# Autodesk Inventor assembly: Additional_Building
(part 2 of 2)
- Flush:52: Walls:1 ↔ Stud_Between_Top_Plate_And_Rafter_3:1
- Flush:53: Walls:1 ↔ Stud_Between_Top_Plate_And_Rafter_3:1
- Mate:71: Walls:1 ↔ Stud_Between_Top_Plate_And_Rafter_4:1
- Flush:54: Walls:1 ↔ Stud_Between_Top_Plate_And_Rafter_4:1
- Flush:55: Walls:1 ↔ Stud_Between_Top_Plate_And_Rafter_4:1
- Mate:72: Walls:1 ↔ Stud_Between_Top_Plate_And_Rafter_5:1
- Flush:56: Walls:1 ↔ Stud_Between_Top_Plate_And_Rafter_5:1
- Flush:57: Walls:1 ↔ Stud_Between_Top_Plate_And_Rafter_5:1
- Mate:73: Walls:1 ↔ Stud_Between_Top_Plate_And_Rafter_6:1
- Flush:58: Walls:1 ↔ Stud_Between_Top_Plate_And_Rafter_6:1
- Flush:59: Walls:1 ↔ Stud_Between_Top_Plate_And_Rafter_6:1
- Mate:74: Walls:1 ↔ Stud_Between_Top_Plate_And_Rafter_7:1
- Flush:60: Walls:1 ↔ Stud_Between_Top_Plate_And_Rafter_7:1
- Flush:61: Walls:1 ↔ Stud_Between_Top_Plate_And_Rafter_7:1
- Mate:75: Walls:1 ↔ Stud_Between_Top_Plate_And_Rafter_8:1
- Flush:62: Walls:1 ↔ Stud_Between_Top_Plate_And_Rafter_8:1
- Flush:63: Walls:1 ↔ Stud_Between_Top_Plate_And_Rafter_8:1
- Mate:76: Walls:1 ↔ Stud_Between_Top_Plate_And_Rafter_9:1
- Mate:77: Truss:1 ↔ Stud_Between_Top_Plate_And_Rafter_9:1
- Flush:64: Walls:1 ↔ Stud_Between_Top_Plate_And_Rafter_9:1
- Mate:78: Walls:1 ↔ Stud_With_Height_41.707_Inches:1
- Mate:79: Truss:1 ↔ Stud_With_Height_41.707_Inches:1
- Mate:80: Stud_Between_Top_Plate_And_Rafter_9:1 ↔ Stud_With_Height_41.707_Inches:1
- Mate:81: Truss:3 ↔ Support_For_Ceiling:1
- Flush:65: Truss:1 ↔ Support_For_Ceiling:1
- Flush:66: Stud_Between_Top_Plate_And_Rafter_1:1 ↔ Support_For_Ceiling:1
- Mate:82: Truss:3 ↔ Support_For_Ceiling:2
- Flush:67: Truss:1 ↔ Support_For_Ceiling:2
- Flush:68: Stud_Between_Top_Plate_And_Rafter_2:1 ↔ Support_For_Ceiling:2
- Mate:83: Truss:3 ↔ Support_For_Ceiling:3
- Flush:69: Truss:1 ↔ Support_For_Ceiling:3
- Flush:70: Stud_Between_Top_Plate_And_Rafter_3:1 ↔ Support_For_Ceiling:3
- Mate:84: Truss:3 ↔ Support_For_Ceiling:4
- Flush:71: Truss:1 ↔ Support_For_Ceiling:4
- Flush:72: Stud_Between_Top_Plate_And_Rafter_4:1 ↔ Support_For_Ceiling:4
- Mate:85: Truss:3 ↔ Support_For_Ceiling:5
- Flush:73: Truss:1 ↔ Support_For_Ceiling:5
- Flush:74: Stud_Between_Top_Plate_And_Rafter_5:1 ↔ Support_For_Ceiling:5
- Mate:86: Truss:3 ↔ Support_For_Ceiling:6
- Flush:75: Truss:1 ↔ Support_For_Ceiling:6
- Flush:76: Stud_Between_Top_Plate_And_Rafter_6:1 ↔ Support_For_Ceiling:6
- Mate:87: Truss:3 ↔ Support_For_Ceiling:7
- Flush:77: Truss:1 ↔ Support_For_Ceiling:7
- Flush:78: Stud_Between_Top_Plate_And_Rafter_7:1 ↔ Support_For_Ceiling:7
- Mate:88: Truss:3 ↔ Support_For_Ceiling:8
- Flush:79: Truss:1 ↔ Support_For_Ceiling:8
- Flush:80: Stud_Between_Top_Plate_And_Rafter_8:1 ↔ Support_For_Ceiling:8
- Mate:89: Truss:3 ↔ Support_For_Ceiling:9
- Flush:81: Truss:1 ↔ Support_For_Ceiling:9
- Mate:90: Walls:1 ↔ Support_For_Ceiling:9
- Mate:91: Truss:3 ↔ Support_For_Ceiling:10
- Flush:82: Truss:3 ↔ Support_For_Ceiling:10
- Mate:92: Truss:1 ↔ Support_For_Ceiling:10
- Flush:83: OSB_For_Side_And_Back:1 ↔ OSB_For_Side_And_Front:1
- Mate:98: OSB_For_Side_And_Back:1
- Angle:1 (0 deg)
- Mate:99: Truss:3 ↔ Subfascia_With_Dimensions_5.798_x_13.75_Inches:1
- Flush:87: Truss:3 ↔ Subfascia_With_Dimensions_5.798_x_13.75_Inches:1
- Flush:88: Truss:3 ↔ Subfascia_With_Dimensions_5.798_x_13.75_Inches:1
- Mate:100: Truss:4 ↔ Subfascia_With_Dimensions_5.798_x_14.5_Inches:1
- Flush:89: Truss:4 ↔ Subfascia_With_Dimensions_5.798_x_14.5_Inches:1
- Flush:90: Truss:4 ↔ Subfascia_With_Dimensions_5.798_x_14.5_Inches:1
- Mate:101: Truss:2 ↔ OSB_For_Walls_With_Dimensions_48_x_96_Inches:13
- Mate:102: OSB_For_Walls_With_Dimensions_48_x_48_Inches:3 ↔ OSB_For_Walls_With_Dimensions_48_x_96_Inches:13
- Flush:91: Truss:2 ↔ OSB_For_Walls_With_Dimensions_48_x_96_Inches:13
- Mate:103: Truss:2 ↔ OSB_For_Walls_With_Dimensions_20.794_x_48_Inches:1
- Mate:104: OSB_For_Walls_With_Dimensions_48_x_96_Inches:13 ↔ OSB_For_Walls_With_Dimensions_20.794_x_48_Inches:1
- Flush:92: Truss:2 ↔ OSB_For_Walls_With_Dimensions_20.794_x_48_Inches:1
- Mate:105: Truss:16 ↔ OSB_For_Walls_With_Dimensions_20.794_x_96_Inches:1
- Mate:106: OSB_For_Walls_With_Dimensions_48_x_96_Inches:14 ↔ OSB_For_Walls_With_Dimensions_20.794_x_96_Inches:1
- Mate:107: OSB_For_Walls_With_Dimensions_20.794_x_96_Inches:1 ↔ OSB_For_Walls_With_Dimensions_20.794_x_48_Inches:1
- Flush:93 (-6.35 mm): Siding_For_Front_Wall:1 ↔ OSB_For_Walls_With_Dimensions_48_x_96_Inches:8
- Flush:94 (-12.7 mm): Siding_For_Front_Wall:1 ↔ OSB_For_Walls_With_Dimensions_48_x_96_Inches:8
- Mate:108: Siding_For_Front_Wall:1 ↔ OSB_For_Walls_With_Dimensions_48_x_96_Inches:13
- Mate:109: Truss:1 ↔ Fascia_For_Front:1
- Mate:111: OSB_For_Side_And_Back:1 ↔ OSB_For_Side_And_Front:1
- Mate:112: OSB_For_Side_And_Back:1 ↔ OSB_For_Side_And_Front:1
- Mate:113: Walls:1 ↔ OSB_For_Walls_With_Dimensions_48_x_48_Inches:5
- Mate:114: OSB_For_Walls_With_Dimensions_48_x_48_Inches:5 ↔ OSB_For_Side_And_Back:1
- Mate:115: DensGlass_With_Dimensions_60.75_x_12_Inches:4 ↔ OSB_For_Walls_With_Dimensions_48_x_48_Inches:5
- Mate:116: Walls:1 ↔ OSB_For_Walls_With_Dimensions_48_x_85_Inches:1
- Mate:117: OSB_For_Walls_With_Dimensions_48_x_48_Inches:5 ↔ OSB_For_Walls_With_Dimensions_48_x_85_Inches:1
- Mate:118: OSB_For_Walls_With_Dimensions_48_x_85_Inches:1 ↔ OSB_For_Side_And_Back:1
- Mate:119: Walls:1 ↔ OSB_For_Walls_With_Dimensions_48_x_96_Inches:16
- Mate:120: OSB_For_Walls_With_Dimensions_48_x_96_Inches:16 ↔ OSB_For_Walls_With_Dimensions_48_x_48_Inches:5
- Flush:98: OSB_For_Walls_With_Dimensions_48_x_96_Inches:16 ↔ OSB_For_Walls_With_Dimensions_48_x_96_Inches:3
- Mate:121: Walls:1 ↔ OSB_For_Walls_With_Dimensions_37_x_48_Inches:1
- Mate:122: OSB_For_Walls_With_Dimensions_37_x_48_Inches:1 ↔ OSB_For_Walls_With_Dimensions_48_x_85_Inches:1
- Mate:126: Fascia_For_Front:1 ↔ Fascia_For_Side:1
- Flush:104 (-57.3151 mm): Truss:1 ↔ Fascia_For_Back:1
- Flush:105: Fascia_For_Back:1 ↔ Fascia_For_Side:1
- Flush:109: Drip_Edge_For_Back:1 ↔ Fascia_For_Back:1
- Mate:128: Drip_Edge_For_Back:1 ↔ Fascia_For_Back:1
- Mate:131: OSB_For_Walls_With_Dimensions_48_x_96_Inches:16 ↔ OSB_For_Walls_With_Dimensions_37_x_48_Inches:1
- Flush:115: Truss:1 ↔ OSB_For_Rear_Roof:1
- Mate:132: Truss:1 ↔ OSB_For_Rear_Roof:1
- Flush:116: Truss:1 ↔ OSB_For_Rear_Roof:1
- Mate:133 (1.5875 mm): Siding_For_Left_Wall:1 ↔ OSB_For_Walls_With_Dimensions_48_x_96_Inches:16
- Flush:117 (-6.35 mm): Siding_For_Left_Wall:1 ↔ OSB_For_Walls_With_Dimensions_48_x_96_Inches:16
- Mate:134: Siding_For_Left_Wall:1 ↔ Fascia_For_Back:1
- Mate:135 (1.5875 mm): Siding_For_Right_Wall:1 ↔ OSB_For_Walls_With_Dimensions_48_x_96_Inches:17
- Mate:136: Siding_For_Right_Wall:1 ↔ Fascia_For_Back:3
- Flush:118 (-6.35 mm): Siding_For_Right_Wall:1 ↔ OSB_For_Walls_With_Dimensions_37_x_48_Inches:2
- Mate:137: Drip_Edge_For_Back:1 ↔ OSB_For_Rear_Roof:2
- Flush:122: Underlayment_For_Side:1 ↔ OSB_For_Walls_With_Dimensions_37_x_48_Inches:1
- Flush:124: Underlayment_For_Side:2 ↔ Truss:2
- Mate:145: Underlayment_For_Side:2 ↔ OSB_For_Side_And_Top:2
- Flush:125: Underlayment_For_Side:2 ↔ OSB_For_Walls_With_Dimensions_48_x_96_Inches:8
- Mate:146: Underlayment_For_Front:1 ↔ OSB_For_Walls_With_Dimensions_48_x_96_Inches:15
- Flush:126: Underlayment_For_Front:1 ↔ Underlayment_For_Side:2
- Mate:147: Underlayment_For_Front:1 ↔ Truss:2
- Mate:148: OSB_For_Side_And_Top:2 ↔ OSB_For_Roof_With_Dimensions_48_x_48:1
- Mate:149: Truss:19 ↔ OSB_For_Roof_With_Dimensions_48_x_48:1
- Mate:150: OSB_For_Rear_Roof:3 ↔ OSB_For_Roof_With_Dimensions_48_x_48:1
- Mate:151: OSB_For_Rear_Roof:3 ↔ OSB_For_Roof_With_Dimensions_96_x_48:4
- Mate:152: OSB_For_Roof_With_Dimensions_48_x_48:1 ↔ OSB_For_Roof_With_Dimensions_47.416_x_96:1
- Mate:153: Truss:1 ↔ OSB_For_Roof_With_Dimensions_47.416_x_96:1
- Flush:127: Truss:2 ↔ OSB_For_Roof_With_Dimensions_47.416_x_96:1
- Flush:128: OSB_For_Side_And_Back:1 ↔ OSB_For_Rear_Roof:1
- Mate:184: Truss:1 ↔ OSB_For_Side_And_Top:1
- Mate:185: OSB_For_Side_And_Back:1 ↔ OSB_For_Side_And_Top:1
- Flush:151 (25.4 mm): Truss:1 ↔ OSB_For_Side_And_Top:1
- Mate:186: Fascia_For_Front:1 ↔ OSB_For_Roof_With_Dimensions_47.416_x_96:3
- Mate:187: Fascia_For_Side:1
- Angle:2 (90 deg)
- Mate:188: Drip_Edge_For_Back:1 ↔ Leak_Barrier:1
- Flush:153: Leak_Barrier:1 ↔ Fascia_For_Side:1
- Mate:189: Drip_Edge_For_Back:1 ↔ Leak_Barrier:1
- Mate:190: Leak_Barrier:1 ↔ Underlayment_For_Roof_With_Width_48_Inches:1
- Flush:154: Leak_Barrier:1 ↔ Underlayment_For_Roof_With_Width_48_Inches:1
- Mate:191 (-50.8 mm): Leak_Barrier:1 ↔ Underlayment_For_Roof_With_Width_48_Inches:1
- Mate:192: Underlayment_For_Roof_With_Width_48_Inches:1 ↔ Underlayment_For_Roof_With_Width_48_Inches:2
- Flush:155: Underlayment_For_Roof_With_Width_48_Inches:1 ↔ Underlayment_For_Roof_With_Width_48_Inches:2
- Mate:193 (-50.8 mm): Underlayment_For_Roof_With_Width_48_Inches:1 ↔ Underlayment_For_Roof_With_Width_48_Inches:2
- Mate:194: Underlayment_For_Roof_With_Width_48_Inches:2 ↔ Underlayment_For_Roof_With_Width_19.157_Inches:1
- Flush:156: Underlayment_For_Roof_With_Width_48_Inches:2 ↔ Underlayment_For_Roof_With_Width_19.157_Inches:1
- Mate:195 (-50.8 mm): Underlayment_For_Roof_With_Width_48_Inches:2 ↔ Underlayment_For_Roof_With_Width_19.157_Inches:1
- Mate:197 (1.5875 mm): Drip_Edge_For_Side:3 ↔ Fascia_For_Side:1
- Mate:198: Underlayment_For_Roof_With_Width_19.157_Inches:1 ↔ Drip_Edge_For_Side:3
- Mate:199: Leak_Barrier:1 ↔ Drip_Edge_For_Side:3
- Mate:202: Drip_Edge_For_Back:1 ↔ Fascia_For_Side:1
- Flush:157: Underlayment_For_Side:1 ↔ DensGlass_With_Dimensions_60.75_x_12_Inches:4
- Flush:158 (-6.35 mm): Siding_For_Back_Wall:1 ↔ DensGlass_With_Dimensions_60.75_x_12_Inches:2
- Mate:207 (-25.4 mm): Siding_For_Left_Wall:1 ↔ Fascia_For_Front:1
- Mate:208: Drip_Edge_For_Side:4 ↔ Fascia_For_Side:2
- Mate:209: Underlayment_For_Roof_With_Width_19.157_Inches:1 ↔ Drip_Edge_For_Side:4
- Mate:210: Leak_Barrier:1 ↔ Drip_Edge_For_Side:4
- Mate:211: Drip_Edge_For_Side:3 ↔ Drip_Edge_For_Front:1
- Mate:212 (1.5875 mm): Drip_Edge_For_Front:1 ↔ Fascia_For_Front:1
- Mate:213: Drip_Edge_For_Side:3 ↔ Drip_Edge_For_Front:1
- Mate:214: Drip_Edge_For_Side:3 ↔ Starter_Shingle_With_Dimensions_6.5_x_35_Inches:1
- Mate:215 (-19.05 mm): Drip_Edge_For_Side:3 ↔ Starter_Shingle_With_Dimensions_6.5_x_35_Inches:1
- Mate:216 (-28.575 mm): Drip_Edge_For_Side:3 ↔ Starter_Shingle_With_Dimensions_6.5_x_35_Inches:1
- Mate:218: Starter_Shingle_With_Dimensions_6.5_x_35_Inches:1 ↔ Starter_Shingle_With_Dimensions_6.5_x_38_Inches:19
- Flush:159: Starter_Shingle_With_Dimensions_6.5_x_35_Inches:1 ↔ Starter_Shingle_With_Dimensions_6.5_x_38_Inches:19
- Flush:160: Starter_Shingle_With_Dimensions_6.5_x_35_Inches:1 ↔ Starter_Shingle_With_Dimensions_6.5_x_38_Inches:19
- Mate:220: Starter_Shingle_With_Dimensions_6.5_x_32.075_Inches:1 ↔ Starter_Shingle_With_Dimensions_6.5_x_38_Inches:24
- Flush:161: Starter_Shingle_With_Dimensions_6.5_x_32.075_Inches:1 ↔ Starter_Shingle_With_Dimensions_6.5_x_38_Inches:24
- Flush:162: Starter_Shingle_With_Dimensions_6.5_x_32.075_Inches:1 ↔ Starter_Shingle_With_Dimensions_6.5_x_38_Inches:24
- Mate:222 (-76.2 mm): Starter_Shingle_With_Dimensions_6.5_x_35_Inches:1 ↔ Starter_Shingle_With_Dimensions_6.5_x_38_Inches:25
- Flush:163: Starter_Shingle_With_Dimensions_6.5_x_35_Inches:1 ↔ Starter_Shingle_With_Dimensions_6.5_x_38_Inches:25
- Flush:164 (-3.175 mm): Starter_Shingle_With_Dimensions_6.5_x_35_Inches:1 ↔ Starter_Shingle_With_Dimensions_6.5_x_38_Inches:25
- Mate:223: Drip_Edge_For_Front:1 ↔ Starter_Shingle_With_Dimensions_6.5_x_29.875_Inches:1
- Mate:224: Starter_Shingle_With_Dimensions_6.5_x_29.875_Inches:1 ↔ Starter_Shingle_With_Dimensions_6.5_x_38_Inches:27
- Flush:165: Starter_Shingle_With_Dimensions_6.5_x_29.875_Inches:1 ↔ Starter_Shingle_With_Dimensions_6.5_x_38_Inches:27
- Mate:225: Starter_Shingle_With_Dimensions_6.5_x_35_Inches:2 ↔ Starter_Shingle_With_Dimensions_6.5_x_29.875_Inches:1
- Flush:166: Starter_Shingle_With_Dimensions_6.5_x_35_Inches:2 ↔ Starter_Shingle_With_Dimensions_6.5_x_29.875_Inches:1
- Flush:167: Starter_Shingle_With_Dimensions_6.5_x_35_Inches:2 ↔ Starter_Shingle_With_Dimensions_6.5_x_29.875_Inches:1
- Mate:226: Starter_Shingle_With_Dimensions_6.5_x_35_Inches:2 ↔ Starter_Shingle_With_Dimensions_6.5_x_38_Inches:31
- Flush:168: Starter_Shingle_With_Dimensions_6.5_x_35_Inches:2 ↔ Starter_Shingle_With_Dimensions_6.5_x_38_Inches:31
- Flush:169: Starter_Shingle_With_Dimensions_6.5_x_35_Inches:2 ↔ Starter_Shingle_With_Dimensions_6.5_x_38_Inches:31
- Flush:170: Starter_Shingle_With_Dimensions_6.5_x_32.075_Inches:2 ↔ Starter_Shingle_With_Dimensions_6.5_x_38_Inches:36
- Mate:227: Starter_Shingle_With_Dimensions_6.5_x_32.075_Inches:2 ↔ Starter_Shingle_With_Dimensions_6.5_x_38_Inches:36
- Flush:171: Starter_Shingle_With_Dimensions_6.5_x_32.075_Inches:2 ↔ Starter_Shingle_With_Dimensions_6.5_x_38_Inches:36
- Mate:228: Shingle_With_Dimensions_13.25_x_39.375_Inches:1 ↔ Starter_Shingle_With_Dimensions_6.5_x_38_Inches:25
- Flush:172: Starter_Shingle_With_Dimensions_6.5_x_35_Inches:1 ↔ Shingle_With_Dimensions_13.25_x_39.375_Inches:1
- Flush:173: Shingle_With_Dimensions_13.25_x_39.375_Inches:1 ↔ Starter_Shingle_With_Dimensions_6.5_x_38_Inches:25
- Mate:229: Shingle_With_Dimensions_13.25_x_19.45_Inches:1 ↔ Starter_Shingle_With_Dimensions_6.5_x_38_Inches:28
- Mate:230: Shingle_With_Dimensions_13.25_x_19.45_Inches:1 ↔ Shingle_With_Dimensions_13.25_x_39.375_Inches:7
- Flush:174: Shingle_With_Dimensions_13.25_x_19.45_Inches:1 ↔ Shingle_With_Dimensions_13.25_x_39.375_Inches:7
- Flush:175 (142.875 mm): Shingle_With_Dimensions_13.25_x_39.375_Inches:1 ↔ Shingle_With_Dimensions_13.25_x_39.375_Inches:14
- Flush:176 (-152.4 mm): Shingle_With_Dimensions_13.25_x_39.375_Inches:14 ↔ Starter_Shingle_With_Dimensions_6.5_x_38_Inches:25
- Mate:231: Shingle_With_Dimensions_13.25_x_39.375_Inches:1 ↔ Shingle_With_Dimensions_13.25_x_39.375_Inches:14
- Mate:232: Shingle_With_Dimensions_13.25_x_19.45_Inches:1 ↔ Shingle_With_Dimensions_13.25_x_25.45_Inches:1
- Mate:234: Shingle_With_Dimensions_13.25_x_25.45_Inches:1 ↔ Bottom_Of_End_Cap_Of_Intake_Vent:1
- Flush:179 (142.875 mm): Bottom_Of_End_Cap_Of_Intake_Vent:1 ↔ Shingle_With_Dimensions_13.25_x_39.375_Inches:14
- Flush:180: Leak_Barrier:1 ↔ Bottom_Of_End_Cap_Of_Intake_Vent:1
- Flush:181 (3.175 mm): Bottom_Of_End_Cap_Of_Intake_Vent:1 ↔ Intake_Vent:1
- Mate:235: Bottom_Of_End_Cap_Of_Intake_Vent:1 ↔ Intake_Vent:1
- Flush:182: Bottom_Of_End_Cap_Of_Intake_Vent:1 ↔ Intake_Vent:1
- Mate:236: Intake_Vent:1 ↔ Side_Of_End_Cap_For_Intake_Vent:1
- Mate:237: Bottom_Of_End_Cap_Of_Intake_Vent:1 ↔ Side_Of_End_Cap_For_Intake_Vent:1
- Flush:183: Bottom_Of_End_Cap_Of_Intake_Vent:1 ↔ Side_Of_End_Cap_For_Intake_Vent:1
- Mate:238: Side_Of_End_Cap_For_Intake_Vent:1 ↔ Bottom_Of_End_Cap_Of_Intake_Vent:2
- Flush:184: Side_Of_End_Cap_For_Intake_Vent:1 ↔ Bottom_Of_End_Cap_Of_Intake_Vent:2
- Mate:239: Intake_Vent:1 ↔ Bottom_Of_End_Cap_Of_Intake_Vent:2
- Mate:240: Shingle_With_Dimensions_13.25_x_25.45_Inches:1 ↔ Bottom_Of_End_Cap_Of_Intake_Vent:3
- Flush:185: Shingle_With_Dimensions_13.25_x_25.45_Inches:1 ↔ Bottom_Of_End_Cap_Of_Intake_Vent:3
- Flush:186 (142.875 mm): Shingle_With_Dimensions_13.25_x_25.45_Inches:1 ↔ Bottom_Of_End_Cap_Of_Intake_Vent:3
- Mate:241: Intake_Vent:1 ↔ Side_Of_End_Cap_For_Intake_Vent:2
- Mate:242: Bottom_Of_End_Cap_Of_Intake_Vent:3 ↔ Side_Of_End_Cap_For_Intake_Vent:2
- Flush:187: Bottom_Of_End_Cap_Of_Intake_Vent:3 ↔ Side_Of_End_Cap_For_Intake_Vent:2
- Mate:243: Side_Of_End_Cap_For_Intake_Vent:2 ↔ Bottom_Of_End_Cap_Of_Intake_Vent:4
- Mate:244: Intake_Vent:1 ↔ Bottom_Of_End_Cap_Of_Intake_Vent:4
- Flush:188: Side_Of_End_Cap_For_Intake_Vent:2 ↔ Bottom_Of_End_Cap_Of_Intake_Vent:4
- Mate:249: First_Shingle_Over_Intake_Vent_With_Length_28.375_Inches:1 ↔ First_Shingle_Over_Intake_Vent_With_Length_39.375_Inches:1
- Flush:192: First_Shingle_Over_Intake_Vent_With_Length_28.375_Inches:1 ↔ First_Shingle_Over_Intake_Vent_With_Length_39.375_Inches:1
- Mate:251: First_Shingle_Over_Intake_Vent_With_Length_30.45_Inches:1 ↔ First_Shingle_Over_Intake_Vent_With_Length_39.375_Inches:6
- Flush:193: First_Shingle_Over_Intake_Vent_With_Length_30.45_Inches:1 ↔ First_Shingle_Over_Intake_Vent_With_Length_39.375_Inches:6
- Mate:252: First_Shingle_Over_Intake_Vent_With_Length_28.375_Inches:1 ↔ Second_Shingle_Over_Intake_Vent_With_Length_22.375_Inches:1
- Flush:194: First_Shingle_Over_Intake_Vent_With_Length_28.375_Inches:1 ↔ Second_Shingle_Over_Intake_Vent_With_Length_22.375_Inches:1
- Flush:195 (142.875 mm): First_Shingle_Over_Intake_Vent_With_Length_28.375_Inches:1 ↔ Second_Shingle_Over_Intake_Vent_With_Length_22.375_Inches:1
- Mate:253: First_Shingle_Over_Intake_Vent_With_Length_39.375_Inches:1 ↔ Second_Shingle_Over_Intake_Vent_With_Length_39.375_Inches:1
- Mate:254: Second_Shingle_Over_Intake_Vent_With_Length_22.375_Inches:1 ↔ Second_Shingle_Over_Intake_Vent_With_Length_39.375_Inches:1
- Flush:196: Second_Shingle_Over_Intake_Vent_With_Length_22.375_Inches:1 ↔ Second_Shingle_Over_Intake_Vent_With_Length_39.375_Inches:1
- Mate:255: First_Shingle_Over_Intake_Vent_With_Length_30.45_Inches:1 ↔ Second_Shingle_Over_Intake_Vent_With_Length_36.45_Inches:1
- Flush:197 (142.875 mm): First_Shingle_Over_Intake_Vent_With_Length_30.45_Inches:1 ↔ Second_Shingle_Over_Intake_Vent_With_Length_36.45_Inches:1
- Mate:256: Second_Shingle_Over_Intake_Vent_With_Length_36.45_Inches:1 ↔ Second_Shingle_Over_Intake_Vent_With_Length_39.375_Inches:6
- Mate:257: Second_Shingle_Over_Intake_Vent_With_Length_22.375_Inches:1 ↔ Third_Shingle_Over_Intake_Vent_With_Length_39.375_Inches:1
- Flush:198 (142.875 mm): Second_Shingle_Over_Intake_Vent_With_Length_22.375_Inches:1 ↔ Third_Shingle_Over_Intake_Vent_With_Length_39.375_Inches:1
- Flush:199: Second_Shingle_Over_Intake_Vent_With_Length_22.375_Inches:1 ↔ Third_Shingle_Over_Intake_Vent_With_Length_39.375_Inches:1
- Mate:258: Second_Shingle_Over_Intake_Vent_With_Length_36.45_Inches:1 ↔ Third_Shingle_Over_Intake_Vent_With_Length_19.45_Inches:1
- Flush:200: Third_Shingle_Over_Intake_Vent_With_Length_19.45_Inches:1 ↔ Third_Shingle_Over_Intake_Vent_With_Length_39.375_Inches:7
- Mate:259: Third_Shingle_Over_Intake_Vent_With_Length_19.45_Inches:1 ↔ Third_Shingle_Over_Intake_Vent_With_Length_39.375_Inches:7
- Flush:201: Second_Shingle_Over_Intake_Vent_With_Length_22.375_Inches:1 ↔ Third_Shingle_Over_Intake_Vent_With_Length_39.375_Inches:1
- Flush:202: First_Shingle_Over_Intake_Vent_With_Length_28.375_Inches:1 ↔ Shingle_With_Dimensions_13.25_x_39.375_Inches:1
- Mate:263: Shingle_With_Dimensions_13.25_x_25.45_Inches:1 ↔ Shingle_With_Dimensions_13.25_x_39.375_Inches:20
- Flush:203: Shingle_With_Dimensions_13.25_x_25.45_Inches:1 ↔ Shingle_With_Dimensions_13.25_x_39.375_Inches:20
- Mate:264: Shingle_With_Dimensions_13.25_x_19.45_Inches:1 ↔ Shingle_With_Dimensions_13.25_x_25.45_Inches:1
- Flush:205: Shingle_With_Dimensions_13.25_x_39.375_Inches:8 ↔ Third_Shingle_Over_Intake_Vent_With_Length_39.375_Inches:1
- Mate:265: Shingle_With_Dimensions_13.25_x_33.375_Inches:1 ↔ Third_Shingle_Over_Intake_Vent_With_Length_39.375_Inches:1
- Mate:266 (102.8954 mm): Shingle_With_Dimensions_13.25_x_33.375_Inches:1 ↔ Third_Shingle_Over_Intake_Vent_With_Length_39.375_Inches:1
- Mate:267: Shingle_With_Dimensions_13.25_x_39.375_Inches:8 ↔ Shingle_With_Dimensions_13.25_x_39.375_Inches:21
- Mate:268: Shingle_With_Dimensions_13.25_x_33.375_Inches:1 ↔ Shingle_With_Dimensions_13.25_x_39.375_Inches:21
- Flush:206: Shingle_With_Dimensions_13.25_x_39.375_Inches:8 ↔ Third_Shingle_Over_Intake_Vent_With_Length_39.375_Inches:1
- Flush:207: First_Shingle_Over_Intake_Vent_With_Length_28.375_Inches:1 ↔ Second_Shingle_Over_Intake_Vent_With_Length_22.375_Inches:1
- Flush:208: Shingle_With_Dimensions_13.25_x_33.375_Inches:1 ↔ Shingle_With_Dimensions_13.25_x_39.375_Inches:21
- Mate:269: Third_Shingle_Over_Intake_Vent_With_Length_19.45_Inches:1 ↔ Shingle_With_Dimensions_13.25_x_25.45_Inches:2
- Mate:270: Shingle_With_Dimensions_13.25_x_25.45_Inches:2 ↔ Shingle_With_Dimensions_13.25_x_39.375_Inches:26
- Flush:209: Shingle_With_Dimensions_13.25_x_25.45_Inches:2 ↔ Shingle_With_Dimensions_13.25_x_39.375_Inches:26
- Mate:271: Shingle_With_Dimensions_13.25_x_33.375_Inches:1 ↔ Shingle_With_Dimensions_13.25_x_28.375_Inches:1
- Flush:210: Shingle_With_Dimensions_13.25_x_33.375_Inches:1 ↔ Shingle_With_Dimensions_13.25_x_28.375_Inches:1
- Flush:211 (142.875 mm): Shingle_With_Dimensions_13.25_x_33.375_Inches:1 ↔ Shingle_With_Dimensions_13.25_x_28.375_Inches:1
- Mate:272: Shingle_With_Dimensions_13.25_x_39.375_Inches:21 ↔ Shingle_With_Dimensions_13.25_x_39.375_Inches:27
- Mate:273: Shingle_With_Dimensions_13.25_x_28.375_Inches:1 ↔ Shingle_With_Dimensions_13.25_x_39.375_Inches:27
- Flush:212: Shingle_With_Dimensions_13.25_x_28.375_Inches:1 ↔ Shingle_With_Dimensions_13.25_x_39.375_Inches:27
- Mate:274: Shingle_With_Dimensions_13.25_x_25.45_Inches:2 ↔ Shingle_With_Dimensions_13.25_x_30.45_Inches:1
- Flush:213: Shingle_With_Dimensions_13.25_x_30.45_Inches:1 ↔ Shingle_With_Dimensions_13.25_x_39.375_Inches:32
- Flush:214: Shingle_With_Dimensions_13.25_x_25.45_Inches:2 ↔ Shingle_With_Dimensions_13.25_x_30.45_Inches:1
- Mate:275: Shingle_With_Dimensions_13.25_x_28.375_Inches:1 ↔ Shingle_With_Dimensions_13.25_x_22.375_Inches:1
- Flush:215: Shingle_With_Dimensions_13.25_x_28.375_Inches:1 ↔ Shingle_With_Dimensions_13.25_x_22.375_Inches:1
- Flush:216 (142.875 mm): Shingle_With_Dimensions_13.25_x_28.375_Inches:1 ↔ Shingle_With_Dimensions_13.25_x_22.375_Inches:1
- Mate:276: Shingle_With_Dimensions_13.25_x_39.375_Inches:27 ↔ Shingle_With_Dimensions_13.25_x_39.375_Inches:33
- Mate:277: Shingle_With_Dimensions_13.25_x_22.375_Inches:1 ↔ Shingle_With_Dimensions_13.25_x_39.375_Inches:33
- Flush:217: Shingle_With_Dimensions_13.25_x_22.375_Inches:1 ↔ Shingle_With_Dimensions_13.25_x_39.375_Inches:33
- Mate:278: Shingle_With_Dimensions_13.25_x_30.45_Inches:1 ↔ Shingle_With_Dimensions_13.25_x_36.45_Inches:1
- Mate:279: Shingle_With_Dimensions_13.25_x_36.45_Inches:1 ↔ Shingle_With_Dimensions_13.25_x_39.375_Inches:38
- Flush:218: Shingle_With_Dimensions_13.25_x_36.45_Inches:1 ↔ Shingle_With_Dimensions_13.25_x_39.375_Inches:38
- Mate:280: Shingle_With_Dimensions_13.25_x_22.375_Inches:1 ↔ Shingle_With_Dimensions_13.25_x_39.375_Inches:39
- Flush:219: Shingle_With_Dimensions_13.25_x_22.375_Inches:1 ↔ Shingle_With_Dimensions_13.25_x_39.375_Inches:39
- Flush:220 (142.875 mm): Shingle_With_Dimensions_13.25_x_22.375_Inches:1 ↔ Shingle_With_Dimensions_13.25_x_39.375_Inches:39
- Mate:281: Shingle_With_Dimensions_13.25_x_36.45_Inches:1 ↔ Shingle_With_Dimensions_13.25_x_19.45_Inches:2
- Mate:282: Shingle_With_Dimensions_13.25_x_19.45_Inches:2 ↔ Shingle_With_Dimensions_13.25_x_39.375_Inches:45
- Flush:221: Shingle_With_Dimensions_13.25_x_19.45_Inches:2 ↔ Shingle_With_Dimensions_13.25_x_39.375_Inches:45
- Mate:283: Shingle_With_Dimensions_13.25_x_33.375_Inches:2 ↔ Shingle_With_Dimensions_13.25_x_39.375_Inches:39
- Flush:222: Shingle_With_Dimensions_13.25_x_33.375_Inches:2 ↔ Shingle_With_Dimensions_13.25_x_39.375_Inches:39
- Flush:223 (142.875 mm): Shingle_With_Dimensions_13.25_x_33.375_Inches:2 ↔ Shingle_With_Dimensions_13.25_x_39.375_Inches:39
- Mate:284: Shingle_With_Dimensions_13.25_x_39.375_Inches:40 ↔ Shingle_With_Dimensions_13.25_x_39.375_Inches:46
- Mate:285: Shingle_With_Dimensions_13.25_x_33.375_Inches:2 ↔ Shingle_With_Dimensions_13.25_x_39.375_Inches:46
- Flush:224: Shingle_With_Dimensions_13.25_x_33.375_Inches:2 ↔ Shingle_With_Dimensions_13.25_x_39.375_Inches:46
- Mate:286: Shingle_With_Dimensions_13.25_x_19.45_Inches:2 ↔ Shingle_With_Dimensions_13.25_x_25.45_Inches:3
- Mate:287: Shingle_With_Dimensions_13.25_x_25.45_Inches:3 ↔ Shingle_With_Dimensions_13.25_x_39.375_Inches:51
- Flush:225: Shingle_With_Dimensions_13.25_x_25.45_Inches:3 ↔ Shingle_With_Dimensions_13.25_x_39.375_Inches:51
- Mate:288: Shingle_With_Dimensions_13.25_x_33.375_Inches:2 ↔ Shingle_With_Dimensions_13.25_x_28.375_Inches:2
- Flush:226: Shingle_With_Dimensions_13.25_x_33.375_Inches:2 ↔ Shingle_With_Dimensions_13.25_x_28.375_Inches:2
- Flush:227 (142.875 mm): Shingle_With_Dimensions_13.25_x_33.375_Inches:2 ↔ Shingle_With_Dimensions_13.25_x_28.375_Inches:2
- Mate:289: Shingle_With_Dimensions_13.25_x_39.375_Inches:46 ↔ Shingle_With_Dimensions_13.25_x_39.375_Inches:52
- Mate:290: Shingle_With_Dimensions_13.25_x_28.375_Inches:2 ↔ Shingle_With_Dimensions_13.25_x_39.375_Inches:52
- Flush:228: Shingle_With_Dimensions_13.25_x_28.375_Inches:2 ↔ Shingle_With_Dimensions_13.25_x_39.375_Inches:52
- Mate:291: Shingle_With_Dimensions_13.25_x_25.45_Inches:3 ↔ Shingle_With_Dimensions_13.25_x_30.45_Inches:2
- Mate:292: Shingle_With_Dimensions_13.25_x_30.45_Inches:2 ↔ Shingle_With_Dimensions_13.25_x_39.375_Inches:57
- Flush:229: Shingle_With_Dimensions_13.25_x_30.45_Inches:2 ↔ Shingle_With_Dimensions_13.25_x_39.375_Inches:57
- Mate:293: Shingle_With_Dimensions_13.25_x_28.375_Inches:2 ↔ Shingle_With_Dimensions_13.25_x_22.375_Inches:2
- Flush:230: Shingle_With_Dimensions_13.25_x_28.375_Inches:2 ↔ Shingle_With_Dimensions_13.25_x_22.375_Inches:2
- Flush:231 (142.875 mm): Shingle_With_Dimensions_13.25_x_28.375_Inches:2 ↔ Shingle_With_Dimensions_13.25_x_22.375_Inches:2
- Mate:294: Shingle_With_Dimensions_13.25_x_39.375_Inches:52 ↔ Shingle_With_Dimensions_13.25_x_39.375_Inches:58
- Mate:295: Shingle_With_Dimensions_13.25_x_22.375_Inches:2 ↔ Shingle_With_Dimensions_13.25_x_39.375_Inches:58
- Flush:232: Shingle_With_Dimensions_13.25_x_22.375_Inches:2 ↔ Shingle_With_Dimensions_13.25_x_39.375_Inches:58
- Mate:296: Shingle_With_Dimensions_13.25_x_30.45_Inches:2 ↔ Shingle_With_Dimensions_13.25_x_36.45_Inches:2
- Mate:297: Shingle_With_Dimensions_13.25_x_36.45_Inches:2 ↔ Shingle_With_Dimensions_13.25_x_39.375_Inches:63
- Flush:233: Shingle_With_Dimensions_13.25_x_36.45_Inches:2 ↔ Shingle_With_Dimensions_13.25_x_39.375_Inches:63
- Mate:298: Shingle_With_Dimensions_13.25_x_22.375_Inches:2 ↔ Shingle_With_Dimensions_13.25_x_39.375_Inches:64
- Flush:234: Shingle_With_Dimensions_13.25_x_22.375_Inches:2 ↔ Shingle_With_Dimensions_13.25_x_39.375_Inches:64
- Flush:235 (142.875 mm): Shingle_With_Dimensions_13.25_x_22.375_Inches:2 ↔ Shingle_With_Dimensions_13.25_x_39.375_Inches:64
- Mate:299: Shingle_With_Dimensions_13.25_x_36.45_Inches:2 ↔ Shingle_With_Dimensions_13.25_x_19.45_Inches:3
- Mate:300: Shingle_With_Dimensions_13.25_x_19.45_Inches:3 ↔ Shingle_With_Dimensions_13.25_x_39.375_Inches:70
- Flush:236: Shingle_With_Dimensions_13.25_x_19.45_Inches:3 ↔ Shingle_With_Dimensions_13.25_x_39.375_Inches:70
- Mate:301: Shingle_With_Dimensions_13.25_x_33.375_Inches:3 ↔ Shingle_With_Dimensions_13.25_x_39.375_Inches:64
- Flush:237: Shingle_With_Dimensions_13.25_x_33.375_Inches:3 ↔ Shingle_With_Dimensions_13.25_x_39.375_Inches:64
- Flush:238 (142.875 mm): Shingle_With_Dimensions_13.25_x_33.375_Inches:3 ↔ Shingle_With_Dimensions_13.25_x_39.375_Inches:64
- Mate:302: Shingle_With_Dimensions_13.25_x_39.375_Inches:65 ↔ Shingle_With_Dimensions_13.25_x_39.375_Inches:71
- Mate:303: Shingle_With_Dimensions_13.25_x_33.375_Inches:3 ↔ Shingle_With_Dimensions_13.25_x_39.375_Inches:71
- Flush:239: Shingle_With_Dimensions_13.25_x_33.375_Inches:3 ↔ Shingle_With_Dimensions_13.25_x_39.375_Inches:71
- Mate:304: Shingle_With_Dimensions_13.25_x_19.45_Inches:3 ↔ Shingle_With_Dimensions_13.25_x_25.45_Inches:4
- Mate:305: Shingle_With_Dimensions_13.25_x_25.45_Inches:4 ↔ Shingle_With_Dimensions_13.25_x_39.375_Inches:76
- Flush:240: Shingle_With_Dimensions_13.25_x_25.45_Inches:4 ↔ Shingle_With_Dimensions_13.25_x_39.375_Inches:76
- Mate:306: Shingle_With_Dimensions_13.25_x_33.375_Inches:3 ↔ Shingle_With_Dimensions_13.25_x_28.375_Inches:3
- Flush:241: Shingle_With_Dimensions_13.25_x_33.375_Inches:3 ↔ Shingle_With_Dimensions_13.25_x_28.375_Inches:3
- Flush:242 (142.875 mm): Shingle_With_Dimensions_13.25_x_33.375_Inches:3 ↔ Shingle_With_Dimensions_13.25_x_28.375_Inches:3
- Mate:307: Shingle_With_Dimensions_13.25_x_39.375_Inches:71 ↔ Shingle_With_Dimensions_13.25_x_39.375_Inches:77
- Mate:308: Shingle_With_Dimensions_13.25_x_28.375_Inches:3 ↔ Shingle_With_Dimensions_13.25_x_39.375_Inches:77
- Flush:243: Shingle_With_Dimensions_13.25_x_28.375_Inches:3 ↔ Shingle_With_Dimensions_13.25_x_39.375_Inches:77
- Mate:309: Shingle_With_Dimensions_13.25_x_25.45_Inches:4 ↔ Shingle_With_Dimensions_13.25_x_30.45_Inches:3
- Mate:310: Shingle_With_Dimensions_13.25_x_30.45_Inches:3 ↔ Shingle_With_Dimensions_13.25_x_39.375_Inches:82
- Flush:244: Shingle_With_Dimensions_13.25_x_30.45_Inches:3 ↔ Shingle_With_Dimensions_13.25_x_39.375_Inches:82
- Mate:311: Shingle_With_Dimensions_13.25_x_28.375_Inches:3 ↔ Shingle_With_Dimensions_13.25_x_22.375_Inches:3
- Flush:245: Shingle_With_Dimensions_13.25_x_28.375_Inches:3 ↔ Shingle_With_Dimensions_13.25_x_22.375_Inches:3
- Flush:246 (142.875 mm): Shingle_With_Dimensions_13.25_x_28.375_Inches:3 ↔ Shingle_With_Dimensions_13.25_x_22.375_Inches:3
- Mate:312: Shingle_With_Dimensions_13.25_x_39.375_Inches:77 ↔ Shingle_With_Dimensions_13.25_x_39.375_Inches:83
- Mate:313: Shingle_With_Dimensions_13.25_x_22.375_Inches:3 ↔ Shingle_With_Dimensions_13.25_x_39.375_Inches:83
- Flush:247: Shingle_With_Dimensions_13.25_x_22.375_Inches:3 ↔ Shingle_With_Dimensions_13.25_x_39.375_Inches:83
- Mate:314: Shingle_With_Dimensions_13.25_x_30.45_Inches:3 ↔ Shingle_With_Dimensions_13.25_x_36.45_Inches:3
- Mate:315: Shingle_With_Dimensions_13.25_x_36.45_Inches:3 ↔ Shingle_With_Dimensions_13.25_x_39.375_Inches:88
- Flush:248: Shingle_With_Dimensions_13.25_x_36.45_Inches:3 ↔ Shingle_With_Dimensions_13.25_x_39.375_Inches:88
- Mate:316: Shingle_With_Dimensions_13.25_x_22.375_Inches:3 ↔ Shingle_With_Dimensions_13.25_x_39.375_Inches:89
- Flush:249: Shingle_With_Dimensions_13.25_x_22.375_Inches:3 ↔ Shingle_With_Dimensions_13.25_x_39.375_Inches:89
- Flush:250 (142.875 mm): Shingle_With_Dimensions_13.25_x_22.375_Inches:3 ↔ Shingle_With_Dimensions_13.25_x_39.375_Inches:89
- Mate:317: Shingle_With_Dimensions_13.25_x_36.45_Inches:3 ↔ Shingle_With_Dimensions_13.25_x_19.45_Inches:4
- Mate:318: Shingle_With_Dimensions_13.25_x_19.45_Inches:4 ↔ Shingle_With_Dimensions_13.25_x_39.375_Inches:95
- Flush:251: Shingle_With_Dimensions_13.25_x_19.45_Inches:4 ↔ Shingle_With_Dimensions_13.25_x_39.375_Inches:95
- Mate:319: Shingle_With_Dimensions_13.25_x_33.375_Inches:4 ↔ Shingle_With_Dimensions_13.25_x_39.375_Inches:89
- Flush:252: Shingle_With_Dimensions_13.25_x_33.375_Inches:4 ↔ Shingle_With_Dimensions_13.25_x_39.375_Inches:89
- Flush:253 (142.875 mm): Shingle_With_Dimensions_13.25_x_33.375_Inches:4 ↔ Shingle_With_Dimensions_13.25_x_39.375_Inches:89
- Mate:320: Shingle_With_Dimensions_13.25_x_39.375_Inches:90 ↔ Shingle_With_Dimensions_13.25_x_39.375_Inches:96
- Mate:321: Shingle_With_Dimensions_13.25_x_33.375_Inches:4 ↔ Shingle_With_Dimensions_13.25_x_39.375_Inches:96
- Flush:254: Shingle_With_Dimensions_13.25_x_33.375_Inches:4 ↔ Shingle_With_Dimensions_13.25_x_39.375_Inches:96
- Mate:322: Shingle_With_Dimensions_13.25_x_19.45_Inches:4 ↔ Shingle_With_Dimensions_13.25_x_25.45_Inches:5
- Mate:323: Shingle_With_Dimensions_13.25_x_25.45_Inches:5 ↔ Shingle_With_Dimensions_13.25_x_39.375_Inches:101
- Flush:255: Shingle_With_Dimensions_13.25_x_25.45_Inches:5 ↔ Shingle_With_Dimensions_13.25_x_39.375_Inches:101
- Mate:324: Shingle_With_Dimensions_13.25_x_33.375_Inches:4 ↔ Shingle_With_Dimensions_13.25_x_28.375_Inches:4
- Flush:256: Shingle_With_Dimensions_13.25_x_33.375_Inches:4 ↔ Shingle_With_Dimensions_13.25_x_28.375_Inches:4
- Flush:257 (142.875 mm): Shingle_With_Dimensions_13.25_x_33.375_Inches:4 ↔ Shingle_With_Dimensions_13.25_x_28.375_Inches:4
- Mate:325: Shingle_With_Dimensions_13.25_x_39.375_Inches:96 ↔ Shingle_With_Dimensions_13.25_x_39.375_Inches:102
- Mate:326: Shingle_With_Dimensions_13.25_x_28.375_Inches:4 ↔ Shingle_With_Dimensions_13.25_x_39.375_Inches:102
- Flush:258: Shingle_With_Dimensions_13.25_x_28.375_Inches:4 ↔ Shingle_With_Dimensions_13.25_x_39.375_Inches:102
- Mate:327: Shingle_With_Dimensions_13.25_x_25.45_Inches:5 ↔ Shingle_With_Dimensions_13.25_x_30.45_Inches:4
- Mate:328: Shingle_With_Dimensions_13.25_x_30.45_Inches:4 ↔ Shingle_With_Dimensions_13.25_x_39.375_Inches:107
- Flush:259: Shingle_With_Dimensions_13.25_x_30.45_Inches:4 ↔ Shingle_With_Dimensions_13.25_x_39.375_Inches:107
- Mate:329: Shingle_With_Dimensions_13.25_x_28.375_Inches:4 ↔ Shingle_With_Dimensions_13.25_x_22.375_Inches:4
- Flush:260: Shingle_With_Dimensions_13.25_x_28.375_Inches:4 ↔ Shingle_With_Dimensions_13.25_x_22.375_Inches:4
- Flush:261 (142.875 mm): Shingle_With_Dimensions_13.25_x_28.375_Inches:4 ↔ Shingle_With_Dimensions_13.25_x_22.375_Inches:4
- Mate:330: Shingle_With_Dimensions_13.25_x_39.375_Inches:102 ↔ Shingle_With_Dimensions_13.25_x_39.375_Inches:108
- Mate:331: Shingle_With_Dimensions_13.25_x_22.375_Inches:4 ↔ Shingle_With_Dimensions_13.25_x_39.375_Inches:108
- Flush:262: Shingle_With_Dimensions_13.25_x_22.375_Inches:4 ↔ Shingle_With_Dimensions_13.25_x_39.375_Inches:108
- Mate:332: Shingle_With_Dimensions_13.25_x_30.45_Inches:4 ↔ Shingle_With_Dimensions_13.25_x_36.45_Inches:4
- Mate:333: Shingle_With_Dimensions_13.25_x_36.45_Inches:4 ↔ Shingle_With_Dimensions_13.25_x_39.375_Inches:113
- Flush:263: Shingle_With_Dimensions_13.25_x_36.45_Inches:4 ↔ Shingle_With_Dimensions_13.25_x_39.375_Inches:113
- Mate:334: Shingle_With_Dimensions_13.25_x_22.375_Inches:4 ↔ Shingle_With_Dimensions_13.25_x_39.375_Inches:114
- Flush:264: Shingle_With_Dimensions_13.25_x_22.375_Inches:4 ↔ Shingle_With_Dimensions_13.25_x_39.375_Inches:114
- Flush:265 (142.875 mm): Shingle_With_Dimensions_13.25_x_22.375_Inches:4 ↔ Shingle_With_Dimensions_13.25_x_39.375_Inches:114
- Mate:335: Shingle_With_Dimensions_13.25_x_36.45_Inches:4 ↔ Shingle_With_Dimensions_13.25_x_19.45_Inches:5
- Mate:336: Shingle_With_Dimensions_13.25_x_19.45_Inches:5 ↔ Shingle_With_Dimensions_13.25_x_39.375_Inches:120
- Flush:266: Shingle_With_Dimensions_13.25_x_19.45_Inches:5 ↔ Shingle_With_Dimensions_13.25_x_39.375_Inches:120
- Mate:337: Shingle_With_Dimensions_13.25_x_33.375_Inches:5 ↔ Shingle_With_Dimensions_13.25_x_39.375_Inches:114
- Flush:267: Shingle_With_Dimensions_13.25_x_33.375_Inches:5 ↔ Shingle_With_Dimensions_13.25_x_39.375_Inches:114
- Flush:268 (142.875 mm): Shingle_With_Dimensions_13.25_x_33.375_Inches:5 ↔ Shingle_With_Dimensions_13.25_x_39.375_Inches:114
- Mate:338: Shingle_With_Dimensions_13.25_x_39.375_Inches:115 ↔ Shingle_With_Dimensions_13.25_x_39.375_Inches:121
- Mate:339: Shingle_With_Dimensions_13.25_x_33.375_Inches:5 ↔ Shingle_With_Dimensions_13.25_x_39.375_Inches:121
- Flush:269: Shingle_With_Dimensions_13.25_x_33.375_Inches:5 ↔ Shingle_With_Dimensions_13.25_x_39.375_Inches:121
- Mate:340: Shingle_With_Dimensions_13.25_x_19.45_Inches:5 ↔ Shingle_With_Dimensions_13.25_x_25.45_Inches:6
- Mate:341: Shingle_With_Dimensions_13.25_x_25.45_Inches:6 ↔ Shingle_With_Dimensions_13.25_x_39.375_Inches:126
- Flush:270: Shingle_With_Dimensions_13.25_x_25.45_Inches:6 ↔ Shingle_With_Dimensions_13.25_x_39.375_Inches:126
- Mate:342: Shingle_With_Dimensions_13.25_x_33.375_Inches:5 ↔ Shingle_With_Dimensions_13.25_x_28.375_Inches:5
- Flush:271: Shingle_With_Dimensions_13.25_x_33.375_Inches:5 ↔ Shingle_With_Dimensions_13.25_x_28.375_Inches:5
- Flush:272 (142.875 mm): Shingle_With_Dimensions_13.25_x_33.375_Inches:5 ↔ Shingle_With_Dimensions_13.25_x_28.375_Inches:5
- Mate:343: Shingle_With_Dimensions_13.25_x_39.375_Inches:121 ↔ Shingle_With_Dimensions_13.25_x_39.375_Inches:127
- Mate:344: Shingle_With_Dimensions_13.25_x_28.375_Inches:5 ↔ Shingle_With_Dimensions_13.25_x_39.375_Inches:127
- Flush:273: Shingle_With_Dimensions_13.25_x_28.375_Inches:5 ↔ Shingle_With_Dimensions_13.25_x_39.375_Inches:127
- Mate:345: Shingle_With_Dimensions_13.25_x_25.45_Inches:6 ↔ Shingle_With_Dimensions_13.25_x_30.45_Inches:5
- Mate:346: Shingle_With_Dimensions_13.25_x_30.45_Inches:5 ↔ Shingle_With_Dimensions_13.25_x_39.375_Inches:132
- Flush:274: Shingle_With_Dimensions_13.25_x_30.45_Inches:5 ↔ Shingle_With_Dimensions_13.25_x_39.375_Inches:132
- Mate:347: Shingle_With_Dimensions_13.25_x_28.375_Inches:5 ↔ Shingle_With_Dimensions_13.25_x_22.375_Inches:5
- Flush:275: Shingle_With_Dimensions_13.25_x_28.375_Inches:5 ↔ Shingle_With_Dimensions_13.25_x_22.375_Inches:5
- Flush:276 (142.875 mm): Shingle_With_Dimensions_13.25_x_28.375_Inches:5 ↔ Shingle_With_Dimensions_13.25_x_22.375_Inches:5
- Mate:348: Shingle_With_Dimensions_13.25_x_39.375_Inches:127 ↔ Shingle_With_Dimensions_13.25_x_39.375_Inches:133
- Mate:349: Shingle_With_Dimensions_13.25_x_22.375_Inches:5 ↔ Shingle_With_Dimensions_13.25_x_39.375_Inches:133
- Flush:277: Shingle_With_Dimensions_13.25_x_22.375_Inches:5 ↔ Shingle_With_Dimensions_13.25_x_39.375_Inches:133
- Mate:350: Shingle_With_Dimensions_13.25_x_30.45_Inches:5 ↔ Shingle_With_Dimensions_13.25_x_36.45_Inches:5
- Mate:351: Shingle_With_Dimensions_13.25_x_36.45_Inches:5 ↔ Shingle_With_Dimensions_13.25_x_39.375_Inches:138
- Flush:278: Shingle_With_Dimensions_13.25_x_36.45_Inches:5 ↔ Shingle_With_Dimensions_13.25_x_39.375_Inches:138
- Mate:352: Shingle_With_Dimensions_13.25_x_22.375_Inches:5 ↔ Shingle_With_Dimensions_13.25_x_39.375_Inches:139
- Flush:279: Shingle_With_Dimensions_13.25_x_22.375_Inches:5 ↔ Shingle_With_Dimensions_13.25_x_39.375_Inches:139
- Flush:280 (142.875 mm): Shingle_With_Dimensions_13.25_x_22.375_Inches:5 ↔ Shingle_With_Dimensions_13.25_x_39.375_Inches:139
- Mate:353: Shingle_With_Dimensions_13.25_x_36.45_Inches:5 ↔ Shingle_With_Dimensions_13.25_x_19.45_Inches:6
- Mate:354: Shingle_With_Dimensions_13.25_x_19.45_Inches:6 ↔ Shingle_With_Dimensions_13.25_x_39.375_Inches:145
- Flush:281: Shingle_With_Dimensions_13.25_x_19.45_Inches:6 ↔ Shingle_With_Dimensions_13.25_x_39.375_Inches:145
- Mate:355: OSB_For_Side_And_Front:1 ↔ OSB_For_Side_And_Top:1
- Flush:282: Soffit_Strip_Vent:1 ↔ Fascia_For_Front:1
- Flush:283 (25.4 mm): Soffit_Strip_Vent:1 ↔ Fascia_For_Front:1
- Flush:284 (25.4 mm): Soffit_Strip_Vent:1 ↔ Fascia_For_Front:1
